# Autodesk Inventor assembly: 17-0028-0011
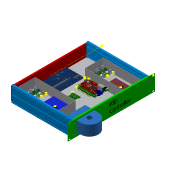
[picture p0: Inventor's stored thumbnail of the model, 180x180]
Saved by Autodesk Inventor 2016 SP2 (Build 200236200, 236)
## iProperties
Created: 2017-10-26
Part Number: 17-0028-0011
Document SubType Name: Assembly
Designer: Daan Giesen
Project: Digital PID Loop
Cost Center: 17-0028
User Status: Work in Progress
Authority: Reichsöllner, Lukas
Description: PID controller
RuleStatus: InUse
Category: -
Company: Universiteit van Amsterdam
BeforeDocSave0: Show Form
Author: Daan Giesen
Title: Digital PID Loop
Revision Number: A
## Documents named in this file (12)
- D:\VaultLocalWorkingFolder\UvA_MT\Projects\2017\17-0028 Digital PID Loop\10_Assemblies\17-0028-0011.iam
- D:\VaultLocalWorkingFolder\UvA_MT\Projects\2017\17-0028 Digital PID Loop\20_3D-Models\17-0028-0012.ipt
- D:\VaultLocalWorkingFolder\UvA_MT\Projects\2017\17-0028 Digital PID Loop\20_3D-Models\17-0028-0003.ipt
- D:\VaultLocalWorkingFolder\UvA_MT\Projects\2017\17-0028 Digital PID Loop\20_3D-Models\17-0028-0013.ipt
- D:\VaultLocalWorkingFolder\UvA_MT\Projects\2017\17-0028 Digital PID Loop\20_3D-Models\17-0028-0014.ipt
- D:\VaultLocalWorkingFolder\UvA_MT\Projects\2017\17-0028 Digital PID Loop\20_3D-Models\Microzed carrier.ipt
- D:\VaultLocalWorkingFolder\UvA_MT\Projects\2017\17-0026-Xray-cell-D.Martin\20_3D-Models\Microzed (No Carrier!).ipt
- D:\VaultLocalWorkingFolder\UvA_MT\Projects\2017\17-0026-Xray-cell-D.Martin\20_3D-Models\8CH_Level_Translator.ipt
- D:\VaultLocalWorkingFolder\UvA_MT\Projects\2017\17-0026-Xray-cell-D.Martin\20_3D-Models\Buffer4Bus_iso_V1.5.ipt
- D:\VaultLocalWorkingFolder\UvA_MT\Projects\2017\17-0026-Xray-cell-D.Martin\20_3D-Models\FAPS.ipt
- D:\VaultLocalWorkingFolder\UvA_MT\Projects\2017\17-0028 Digital PID Loop\20_3D-Models\17-0028-0075.iam
- D:\VaultLocalWorkingFolder\UvA_MT\Projects\2017\17-0028 Digital PID Loop\20_3D-Models\17-0028-0046.iam
## Components (17 placed, 11 different names)
1. 17-0028-0075:1 [sub-assembly] — Mate:29, Mate:30, Mate:31, Mate:32, Mate:33, Mate:34, Mate:35, Mate:36, Mate:47, Mate:48
2. 8CH_Level_Translator:2 — Mate:48
3. Buffer4Bus_iso_V1.5:2 — Mate:46, Mate:47
4. FAPS:7 — Mate:40, Flush:2
5. Microzed (No Carrier!):2
6. 17-0028-0012:1 — Mate:6, Mate:11, Mate:12, Mate:30, Mate:31, Mate:44, Mate:45
7. 17-0028-0012:2 — Mate:5, Mate:13, Mate:14, Mate:32, Mate:38, Mate:39, Mate:42, Mate:43
8. 17-0028-0003:1 — Mate:36, Mate:37, Flush:1
9. 17-0028-0013:1 — Mate:5, Mate:13, Mate:14
10. 17-0028-0014:1 — Mate:6, Mate:11, Mate:12
11. FAPS:8
12. FAPS:9
13. FAPS:10
14. Microzed carrier:1 — Mate:29
15. FAPS:11 — Mate:39, Mate:40, Mate:41, Flush:2, Flush:3
16. FAPS:12 — Mate:38, Mate:41, Flush:3
17. 17-0028-0046:1 [sub-assembly] — Mate:33, Mate:34, Mate:35, Mate:37, Flush:1, Mate:42, Mate:43, Mate:44, Mate:45, Mate:46
## Relationships (44: Mate 40, Flush 3, Angle 1)
- Mate:5: 17-0028-0012:2 ↔ 17-0028-0013:1
- Mate:6: 17-0028-0012:1 ↔ 17-0028-0014:1
- [Mate] (10 mm): FAPS:7 ↔ 17-0028-0012:2
- [Mate] (10 mm): 17-0028-0012:1 ↔ FAPS:10
- [Mate] (10 mm): 17-0028-0012:1 ↔ FAPS:8
- [Mate] (10 mm): 17-0028-0012:1 ↔ FAPS:9
- Mate:11 (10 mm): 17-0028-0012:1 ↔ 17-0028-0014:1
- Mate:12 (10 mm): 17-0028-0012:1 ↔ 17-0028-0014:1
- Mate:13 (10 mm): 17-0028-0012:2 ↔ 17-0028-0013:1
- Mate:14 (1 mm): 17-0028-0012:2 ↔ 17-0028-0013:1
- [Mate] (20 mm): FAPS:7 ↔ 17-0028-0012:2
- [Mate] (10 mm): FAPS:7 ↔ 17-0028-0012:2
- [Mate] (10 mm): 17-0028-0012:1 ↔ FAPS:10
- [Mate] (10 mm): 17-0028-0012:1 ↔ FAPS:8
- [Mate] (10 mm): 17-0028-0012:1 ↔ FAPS:9
- [Mate] (5 mm): 17-0028-0012:1 ↔ FAPS:10
- [Mate] (5 mm): FAPS:8 ↔ FAPS:10
- [Mate] (5 mm): FAPS:8 ↔ FAPS:9
- [Mate]: Microzed (No Carrier!):2 ↔ Microzed carrier:1
- [Mate]: Microzed (No Carrier!):2 ↔ Microzed carrier:1
- [Angle] (0 deg): Microzed (No Carrier!):2 ↔ Microzed carrier:1
- Mate:29 (20 mm): 17-0028-0075:1 ↔ Microzed carrier:1
- Mate:30: 17-0028-0075:1 ↔ 17-0028-0012:1
- Mate:31: 17-0028-0075:1 ↔ 17-0028-0012:1
- Mate:32: 17-0028-0075:1 ↔ 17-0028-0012:2
- Mate:33 (5 mm): 17-0028-0075:1 ↔ 17-0028-0046:1
- Mate:34: 17-0028-0075:1 ↔ 17-0028-0046:1
- Mate:35: 17-0028-0075:1 ↔ 17-0028-0046:1
- Mate:36: 17-0028-0075:1 ↔ 17-0028-0003:1
- Mate:37 (10 mm): 17-0028-0003:1 ↔ 17-0028-0046:1
- Flush:1 (-50 mm): 17-0028-0003:1 ↔ 17-0028-0046:1
- Mate:38 (10 mm): 17-0028-0012:2 ↔ FAPS:12
- Mate:39 (10 mm): 17-0028-0012:2 ↔ FAPS:11
- Mate:40: FAPS:7 ↔ FAPS:11
- Mate:41: FAPS:11 ↔ FAPS:12
- Flush:2: FAPS:7 ↔ FAPS:11
- Flush:3: FAPS:11 ↔ FAPS:12
- Mate:42 (10 mm): 17-0028-0012:2 ↔ 17-0028-0046:1
- Mate:43 (10 mm): 17-0028-0012:2 ↔ 17-0028-0046:1
- Mate:44 (10 mm): 17-0028-0012:1 ↔ 17-0028-0046:1
- Mate:45 (10 mm): 17-0028-0012:1 ↔ 17-0028-0046:1
- Mate:46 (10 mm): Buffer4Bus_iso_V1.5:2 ↔ 17-0028-0046:1
- Mate:47 (10 mm): 17-0028-0075:1 ↔ Buffer4Bus_iso_V1.5:2
- Mate:48 (10 mm): 17-0028-0075:1 ↔ 8CH_Level_Translator:2
